# Autodesk Inventor assembly: date-counter
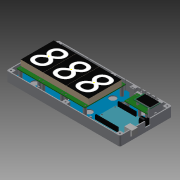
[picture p0: Inventor's stored thumbnail of the model, 180x180]
Saved by Autodesk Inventor 2015 (Build 190159000, 159)
## iProperties
Created: 2016-04-26
Part Number: date-counter
Document SubType Name: Assembly
Designer: yamashita1
Author: yamashita1
## Documents named in this file (6)
- Z:\cygwin\project\date-counter\trunk\date-counter.iam
- Z:\cygwin\project\date-counter\trunk\Big7seg.ipt
- Z:\cygwin\project\date-counter\trunk\Arduino UNO.ipt
- Z:\cygwin\project\date-counter\trunk\LCD-RTC.ipt
- Z:\cygwin\project\date-counter\trunk\top-cover.ipt
- Z:\cygwin\project\date-counter\trunk\bottom-cover.ipt
## Components (7 placed, 5 different names)
1. bottom-cover:1 — メイト:1, メイト:2
2. Big7seg:1
3. Big7seg:2
4. Big7seg:3
5. Arduino UNO:1 — メイト:2
6. LCD-RTC:1 — メイト:1
7. top-cover:1
## Relationships (2: Mate 2)
- メイト:1 [Mate]: bottom-cover:1 ↔ LCD-RTC:1
- メイト:2 [Mate]: bottom-cover:1 ↔ Arduino UNO:1
